# Autodesk Inventor assembly: 40-tooth Gear Assembly
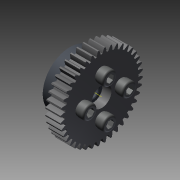
[picture p0: Inventor's stored thumbnail of the model, 180x180]
Saved by Autodesk Inventor 2015 (Build 190159000, 159)
## iProperties
Created: 2015-09-29
Part Number: 40-tooth Gear Assembly
Document SubType Name: Assembly
Designer: Jing-Chen
Author: Jing-Chen
## Documents named in this file (4)
- C:\Users\Jing-Chen\Desktop\Bionic Hybrids 2016\Bionic-Hybrids\CAD\General\40-tooth Gear Assembly.iam
- C:\Users\Jing-Chen\Desktop\Bionic Hybrids 2016\Bionic-Hybrids\Stock\Gear-40 tooth - 731901.ipt
- C:\Users\Jing-Chen\Desktop\Bionic Hybrids 2016\Bionic-Hybrids\Stock\Shaft Collar-Setscrew, Axle, Mountable - 739172.iam
- C:\Users\Jing-Chen\Desktop\Bionic Hybrids 2016\Bionic-Hybrids\Stock\Screw 0.5in - 739097.ipt
## Components (6 placed, 3 different names)
1. Gear-40 tooth - 731901:1 — Mate:1, Mate:2, Mate:3, Mate:4, Mate:5, Mate:6, Mate:7, Mate:8, Mate:9, Mate:10, Mate:11
2. Shaft Collar-Setscrew, Axle, Mountable - 739172:1 [sub-assembly] — Mate:1, Mate:2, Mate:3
3. Screw 0.5in - 739097:1 — Mate:4, Mate:9
4. Screw 0.5in - 739097:2 — Mate:7, Mate:10
5. Screw 0.5in - 739097:3 — Mate:6, Mate:8
6. Screw 0.5in - 739097:4 — Mate:5, Mate:11
## Relationships (11: Mate 11)
- Mate:1: Gear-40 tooth - 731901:1 ↔ Shaft Collar-Setscrew, Axle, Mountable - 739172:1
- Mate:2: Gear-40 tooth - 731901:1 ↔ Shaft Collar-Setscrew, Axle, Mountable - 739172:1
- Mate:3: Gear-40 tooth - 731901:1 ↔ Shaft Collar-Setscrew, Axle, Mountable - 739172:1
- Mate:4: Gear-40 tooth - 731901:1 ↔ Screw 0.5in - 739097:1
- Mate:5: Gear-40 tooth - 731901:1 ↔ Screw 0.5in - 739097:4
- Mate:6: Gear-40 tooth - 731901:1 ↔ Screw 0.5in - 739097:3
- Mate:7: Gear-40 tooth - 731901:1 ↔ Screw 0.5in - 739097:2
- Mate:8: Gear-40 tooth - 731901:1 ↔ Screw 0.5in - 739097:3
- Mate:9: Gear-40 tooth - 731901:1 ↔ Screw 0.5in - 739097:1
- Mate:10: Gear-40 tooth - 731901:1 ↔ Screw 0.5in - 739097:2
- Mate:11: Gear-40 tooth - 731901:1 ↔ Screw 0.5in - 739097:4
